# Autodesk Inventor assembly: MX-106_with_bearing_MIR
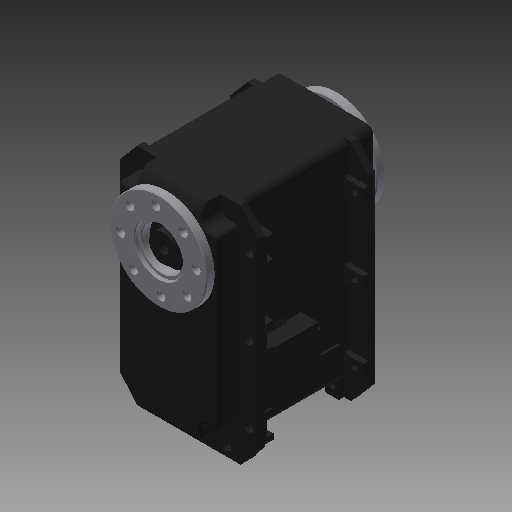
[picture p0: Inventor's stored thumbnail of the model, 512x512]
Saved by Autodesk Inventor 2018 (Build 220112000, 112)
## iProperties
Created: 2015-05-09
Part Number: MX-106_with_bearing_MIR
Document SubType Name: Assembly
Designer: bitbots
Mass: 87.7237 g
Surface Area: 191.727 cm^2
Volume: 87.7237 cm^3
Density: 1 g/cm^3
Author: bitbots
## Documents named in this file (4)
- C:\Users\bitbots\Desktop\bitbots_hardware\wolfgang\assembly\motors\MX106\MX-106_with_bearing_MIR.iam
- C:\Users\bitbots\Desktop\bitbots_hardware\wolfgang\assembly\motors\MX106\MX-106_MIR.ipt
- C:\Users\bitbots\Desktop\bitbots_hardware\wolfgang\assembly\motors\MX64\HN05-N101_MIR1.ipt
- C:\Users\bitbots\Desktop\bitbots_hardware\wolfgang\assembly\motors\MX64\HN05-i1_MIR1.ipt
## Components (3 placed, 3 different names)
1. MX-106_MIR:1 — Rotational:1, Rotational:2
2. HN05-N101_MIR1:1 — Rotational:1
3. HN05-i1_MIR1:1 — Rotational:2
## Relationships (2: RevoluteJoint 2)
- Rotational:1 [RevoluteJoint] (-7 mm): MX-106_MIR:1 ↔ HN05-N101_MIR1:1
- Rotational:2 [RevoluteJoint]: MX-106_MIR:1 ↔ HN05-i1_MIR1:1
